# Autodesk Inventor assembly: base_const_al
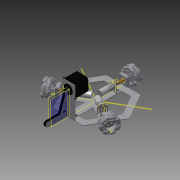
[picture p0: Inventor's stored thumbnail of the model, 180x180]
Saved by Autodesk Inventor 2015 (Build 190159000, 159)
## iProperties
Created: 2015-04-17
Part Number: base_const_al
Document SubType Name: Assembly
Designer: Marcin
Author: Marcin
## Documents named in this file (4)
- C:\Users\Kuba\Dysk Google\synergia\Synergolf\model\GOLF\base_const_al.iam
- C:\Users\Kuba\Dysk Google\synergia\Synergolf\model\GOLF\base_constr.ipt
- C:\Users\Kuba\Dysk Google\synergia\Synergolf\model\GOLF\mot_wheel.iam
- C:\Users\Kuba\Dysk Google\synergia\Synergolf\model\GOLF\stepper_large_all.iam
## Components (5 placed, 3 different names)
1. base_constr:1 — Zestawiający:1, Zestawiający:2, Równoległy:1, Zestawiający:3, Zestawiający:4, Zestawiający:5, Zestawiający:6, Kąt:1, Zestawiający:7, Kąt:2, Zestawiający:8, Kąt:3, Równoległy:2, Równoległy:3, Równoległy:4, Zestawiający:12, Równoległy:6
2. mot_wheel:1 [sub-assembly] — Zestawiający:3, Zestawiający:10, Równoległy:2
3. mot_wheel:2 [sub-assembly] — Zestawiający:4, Zestawiający:11, Równoległy:3
4. mot_wheel:3 [sub-assembly] — Zestawiający:5, Zestawiający:9, Równoległy:4
5. stepper_large_all:1 [sub-assembly] — Zestawiający:12, Równoległy:5, Równoległy:6
## Relationships (21: Mate 12, Flush 6, Angle 3)
- Zestawiający:1 [Mate]: base_constr:1
- Zestawiający:2 [Mate]: base_constr:1
- Równoległy:1 [Flush]: base_constr:1
- Zestawiający:3 [Mate]: base_constr:1 ↔ mot_wheel:1
- Zestawiający:4 [Mate]: base_constr:1 ↔ mot_wheel:2
- Zestawiający:5 [Mate]: base_constr:1 ↔ mot_wheel:3
- Zestawiający:6 [Mate]: base_constr:1
- Kąt:1 [Angle] (0 deg): base_constr:1
- Zestawiający:7 [Mate]: base_constr:1
- Kąt:2 [Angle] (0 deg): base_constr:1
- Zestawiający:8 [Mate]: base_constr:1
- Kąt:3 [Angle] (0 deg): base_constr:1
- Zestawiający:9 [Mate]: mot_wheel:3
- Zestawiający:10 [Mate]: mot_wheel:1
- Zestawiający:11 [Mate]: mot_wheel:2
- Równoległy:2 [Flush]: base_constr:1 ↔ mot_wheel:1
- Równoległy:3 [Flush]: base_constr:1 ↔ mot_wheel:2
- Równoległy:4 [Flush]: base_constr:1 ↔ mot_wheel:3
- Zestawiający:12 [Mate]: base_constr:1 ↔ stepper_large_all:1
- Równoległy:5 [Flush]: stepper_large_all:1
- Równoległy:6 [Flush]: base_constr:1 ↔ stepper_large_all:1
